# Autodesk Inventor assembly: SCS12UU
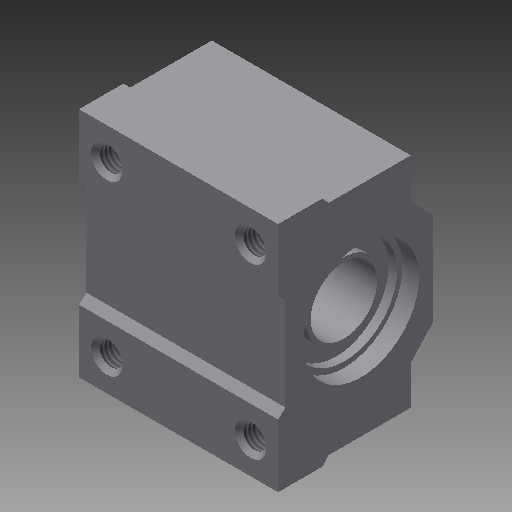
[picture p0: Inventor's stored thumbnail of the model, 512x512]
Saved by Autodesk Inventor 2018 (Build 220112000, 112)
## iProperties
Created: 2018-07-23
Part Number: SCS12UU
Material: Genérico
Document SubType Name: Assembly
Designer: Usuario
Mass: 29.7863 g
Surface Area: 169.387 cm^2
Volume: 29.7863 cm^3
Density: 1 g/cm^3
Author: Usuario
## Documents named in this file (4)
- C:\Users\Usuario\Desktop\pecas_3d-20180530T120808Z-001\pecas_3d\SCS12UU.iam
- C:\Users\Usuario\Desktop\pecas_3d-20180530T120808Z-001\pecas_3d\rolamento_linear_lm12uu.iam.ipt
- C:\Users\Usuario\Desktop\pecas_3d-20180530T120808Z-001\pecas_3d\PilowBlockFechado.ipt
- rolamento_linear_lm12uu.iam
## Components (2 placed, 2 different names)
1. rolamento_linear_lm12uu.iam:1 — Coincidência:1, Alinhamento:1
2. PilowBlockFechado:1 — Coincidência:1, Alinhamento:1
## Relationships (2: Mate 1, Flush 1)
- Coincidência:1 [Mate]: rolamento_linear_lm12uu.iam:1 ↔ PilowBlockFechado:1
- Alinhamento:1 [Flush] (3 mm): rolamento_linear_lm12uu.iam:1 ↔ PilowBlockFechado:1
